# Autodesk Inventor assembly: シリンダ
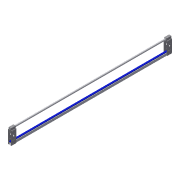
[picture p0: Inventor's stored thumbnail of the model, 180x180]
Saved by Autodesk Inventor 2019.4 (Build 234330000, 330)
## iProperties
Created: 2018-08-09
Part Number: シリンダ
Document SubType Name: Assembly
Designer: Owner
Mass: 175.735 g
Surface Area: 1673.95 cm^2
Volume: 175.735 cm^3
Density: 1 g/cm^3
Author: Owner
## Documents named in this file (6)
- E:\ロボ研\キャチロボ\キャチロボ2019\CADdata\アーム2019\2019HDarm\シリンダ.iam
- E:\ロボ研\キャチロボ\キャチロボ2019\CADdata\アーム2019\2019HDarm\□15.ipt
- E:\ロボ研\キャチロボ\キャチロボ2019\CADdata\アーム2019\2019HDarm\フレキラック.ipt
- E:\ロボ研\キャチロボ\キャチロボ2019\CADdata\アーム2019\2019HDarm\φ10棒.ipt
- E:\ロボ研\キャチロボ\キャチロボ2019\CADdata\アーム2019\2019HDarm\先側板alt.ipt
- E:\ロボ研\キャチロボ\キャチロボ2019\CADdata\アーム2019\2019HDarm\締めつけ肉.ipt
## Components (9 placed, 5 different names)
1. □15:1 — リジッド:4, リジッド:8, リジッド:9, メイト:2
2. フレキラック:1 — リジッド:9
3. φ10棒:1 — リジッド:2, リジッド:7, メイト:1
4. 先側板alt:3 — リジッド:3
5. 先側板alt:4 — リジッド:1, リジッド:4
6. 先側板alt:1 — リジッド:6, リジッド:8
7. 締めつけ肉:1 — リジッド:5, リジッド:6, リジッド:7
8. 先側板alt:2 — リジッド:5
9. 締めつけ肉:2 — リジッド:1, リジッド:2, リジッド:3
## Relationships (11: WeldJoint 9, Mate 2)
- リジッド:1 [WeldJoint]: 先側板alt:4 ↔ 締めつけ肉:2
- リジッド:2 [WeldJoint]: φ10棒:1 ↔ 締めつけ肉:2
- リジッド:3 [WeldJoint]: 先側板alt:3 ↔ 締めつけ肉:2
- リジッド:4 [WeldJoint]: □15:1 ↔ 先側板alt:4
- リジッド:5 [WeldJoint]: 締めつけ肉:1 ↔ 先側板alt:2
- リジッド:6 [WeldJoint]: 先側板alt:1 ↔ 締めつけ肉:1
- リジッド:7 [WeldJoint]: φ10棒:1 ↔ 締めつけ肉:1
- リジッド:8 [WeldJoint]: □15:1 ↔ 先側板alt:1
- リジッド:9 [WeldJoint]: □15:1 ↔ フレキラック:1
- メイト:1 [Mate]: φ10棒:1
- メイト:2 [Mate]: □15:1
